# Autodesk Inventor assembly: Asem
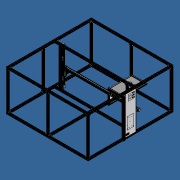
[picture p0: Inventor's stored thumbnail of the model, 180x180]
Saved by Autodesk Inventor 2020 (Build 240168000, 168)
## iProperties
Created: 2021-02-24
Part Number: Asem
Document SubType Name: Assembly
Designer: magnarecta
Author: magnarecta
## Documents named in this file (8)
- D:\Document\Github\Eto_Project\Hardware\Asem\Asem.iam
- D:\Document\Github\Eto_Project\Hardware\Asem\CCM_Unit.iam
- D:\Document\Github\Eto_Project\Hardware\Asem\Display_Unit.iam
- D:\Document\Github\Eto_Project\Hardware\Parts\Meviy\Controller_Panel.ipt
- D:\Document\Github\Eto_Project\Hardware\Parts\Grabcad\ac-power-switch-assembly-1.snapshot.2\AC Power Switch Assy.iam
- D:\Document\Github\Eto_Project\Hardware\Parts\Grabcad\mean-well-lrs-350-24-1.snapshot.3\meanwell_lrs-350-24_UPDATED.ipt
- D:\Document\Github\Eto_Project\Hardware\Parts\Grabcad\nema-23-stepper-motors-driver-1.snapshot.7\DM542T Digital Stepper Drive.ipt
- D:\Document\Github\Eto_Project\Hardware\Asem\FRAMES\FramesEto_Project.iam
## Components (9 placed, 7 different names)
1. Display_Unit:1 [sub-assembly] — メイト:39
2. FramesEto_Project:1 [sub-assembly] — メイト:38, フラッシュ:62, フラッシュ:63, メイト:40, メイト:41, メイト:42, メイト:46
3. CCM_Unit:2 [sub-assembly] — メイト:38, フラッシュ:62, フラッシュ:63, メイト:39
4. Controller_Panel:2 — メイト:40, メイト:41, メイト:42, メイト:43, 角度:1, メイト:44, メイト:45, 角度:2, 挿入:1, 挿入:2, メイト:46
5. meanwell_lrs-350-24_UPDATED:2 — メイト:43, 角度:1
6. AC Power Switch Assy:3 [sub-assembly] — メイト:44, 挿入:1, 挿入:2
7. DM542T Digital Stepper Drive:1 — メイト:45, 角度:2
8. DM542T Digital Stepper Drive:2
9. DM542T Digital Stepper Drive:3
## Component patterns: (3 elements, first: DM542T Digital Stepper Drive:1)
## Relationships (15: Mate 9, Flush 2, Angle 2, Insert 2)
- メイト:38 [Mate] (2 mm): FramesEto_Project:1 ↔ CCM_Unit:2
- フラッシュ:62 [Flush] (-5 mm): FramesEto_Project:1 ↔ CCM_Unit:2
- フラッシュ:63 [Flush] (5 mm): FramesEto_Project:1 ↔ CCM_Unit:2
- メイト:39 [Mate] (5 mm): Display_Unit:1 ↔ CCM_Unit:2
- メイト:40 [Mate]: FramesEto_Project:1 ↔ Controller_Panel:2
- メイト:41 [Mate]: FramesEto_Project:1 ↔ Controller_Panel:2
- メイト:42 [Mate]: FramesEto_Project:1 ↔ Controller_Panel:2
- メイト:43 [Mate]: Controller_Panel:2 ↔ meanwell_lrs-350-24_UPDATED:2
- 角度:1 [Angle] (0 deg): Controller_Panel:2 ↔ meanwell_lrs-350-24_UPDATED:2
- メイト:44 [Mate]: Controller_Panel:2 ↔ AC Power Switch Assy:3
- メイト:45 [Mate]: Controller_Panel:2 ↔ DM542T Digital Stepper Drive:1
- 角度:2 [Angle] (90 deg): Controller_Panel:2 ↔ DM542T Digital Stepper Drive:1
- 挿入:1 [Insert]: Controller_Panel:2 ↔ AC Power Switch Assy:3
- 挿入:2 [Insert]: Controller_Panel:2 ↔ AC Power Switch Assy:3
- メイト:46 [Mate]: FramesEto_Project:1 ↔ Controller_Panel:2
